# Autodesk Inventor assembly: Canister.assembly
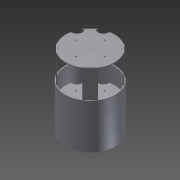
[picture p0: Inventor's stored thumbnail of the model, 180x180]
Saved by Autodesk Inventor 2011 (Build 150239000, 239)
## iProperties
Created: 2011-01-27
Part Number: Canister.assembly
Document SubType Name: Assembly
Designer: Physics Student
Author: Physics Student
## Documents named in this file (4)
- C:\Users\Physics Student\Documents\My Dropbox\RockSAT-X 2011 RexSAT\capsule-launcher.design\Canister.assembly.iam
- C:\Users\Physics Student\Documents\My Dropbox\RockSAT-X 2011 RexSAT\capsule-launcher.design\Deck.ipt
- C:\Users\Physics Student\Documents\My Dropbox\RockSAT-X 2011 RexSAT\capsule-launcher.design\longeron.ipt
- C:\Users\Physics Student\Documents\My Dropbox\RockSAT-X 2011 RexSAT\capsule-launcher.design\skin.25.ipt
## Components (10 placed, 3 different names)
1. Deck:1 — Mate:1, Mate:2, Mate:3
2. Deck:2 — Mate:1, Mate:2, Mate:3, Mate:4, Flush:1, Mate:6, Flush:2, Mate:7, Flush:3, Mate:8, Flush:4
3. longeron:1 — Mate:4, Flush:1, Mate:5, Mate:13, Mate:14
4. longeron:2 — Mate:6, Flush:2, Mate:9, Mate:15, Mate:16
5. longeron:3 — Mate:7, Flush:3, Mate:10, Mate:17, Mate:18
6. longeron:4 — Mate:8, Flush:4, Mate:11, Mate:12, Mate:19
7. skin.25:1 — Mate:12, Mate:13, Flush:7
8. skin.25:2 — Mate:16, Mate:17, Flush:5, Flush:6
9. skin.25:3 — Mate:18, Mate:19, Flush:5, Flush:7
10. skin.25:4 — Mate:14, Mate:15, Flush:6
## Relationships (26: Mate 19, Flush 7)
- Mate:1 (304.8 mm): Deck:1 ↔ Deck:2
- Mate:2: Deck:1 ↔ Deck:2
- Mate:3: Deck:1 ↔ Deck:2
- Mate:4: Deck:2 ↔ longeron:1
- Flush:1: Deck:2 ↔ longeron:1
- Mate:5: longeron:1
- Mate:6: Deck:2 ↔ longeron:2
- Flush:2: Deck:2 ↔ longeron:2
- Mate:7: Deck:2 ↔ longeron:3
- Flush:3: Deck:2 ↔ longeron:3
- Mate:8: Deck:2 ↔ longeron:4
- Flush:4: Deck:2 ↔ longeron:4
- Mate:9: longeron:2
- Mate:10: longeron:3
- Mate:11: longeron:4
- Mate:12: longeron:4 ↔ skin.25:1
- Mate:13: longeron:1 ↔ skin.25:1
- Mate:14: longeron:1 ↔ skin.25:4
- Mate:15: longeron:2 ↔ skin.25:4
- Mate:16: longeron:2 ↔ skin.25:2
- Mate:17: longeron:3 ↔ skin.25:2
- Mate:18: longeron:3 ↔ skin.25:3
- Mate:19: longeron:4 ↔ skin.25:3
- Flush:5: skin.25:2 ↔ skin.25:3
- Flush:6: skin.25:2 ↔ skin.25:4
- Flush:7: skin.25:1 ↔ skin.25:3
